# Autodesk Inventor assembly: Motor
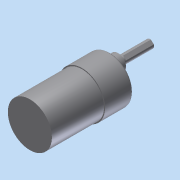
[picture p0: Inventor's stored thumbnail of the model, 180x180]
Saved by Autodesk Inventor 2012 (Build 160160000, 160)
## iProperties
Created: 2011-10-28
Part Number: Motor
Document SubType Name: Assembly
Designer: Kyle
Author: Kyle
## Documents named in this file (3)
- C:\Users\Kyle\Documents\Inventor\2011-12 FTC\Parts\Motor.iam
- C:\Users\Kyle\Documents\Inventor\2011-12 FTC\Parts\Motorbase.ipt
- C:\Users\Kyle\Documents\Inventor\2011-12 FTC\Parts\Motoraxle.ipt
## Components (2 placed, 2 different names)
1. Motorbase:1 — Mate:1, Tangent:1
2. Motoraxle:1 — Mate:1, Tangent:1
## Relationships (2: Mate 1, Tangent 1)
- Mate:1: Motorbase:1 ↔ Motoraxle:1
- Tangent:1: Motorbase:1 ↔ Motoraxle:1
